# Autodesk Inventor assembly: Shooter
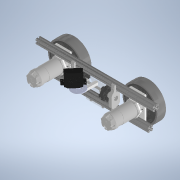
[picture p0: Inventor's stored thumbnail of the model, 180x180]
Saved by Autodesk Inventor 2021 (Build 250183000, 183)
## iProperties
Created: 2021-05-22
Part Number: Shooter
Document SubType Name: Assembly
Designer: sami8
Author: sami8
## Documents named in this file (24)
- C:\Users\sami8\Documents\FTC 2021\CAD\Shooter\Shooter.iam
- C:\Users\sami8\Documents\FTC 2021\CAD\FloorRoller\REV-41-1097.ipt
- C:\Users\sami8\Documents\FTC 2021\CAD\FloorRoller\REV-41-1363.ipt
- C:\Users\sami8\Documents\FTC 2021\CAD\Shooter\ServoArm.ipt
- C:\Users\sami8\Documents\FTC 2021\CAD\FloorRoller\REV-41-1123.ipt
- C:\Users\sami8\Documents\FTC 2021\CAD\Shooter\REV-41-1607.ipt
- C:\Users\sami8\Documents\FTC 2021\CAD\Shooter\REV-41-1608.ipt
- C:\Users\sami8\Documents\FTC 2021\CAD\Shooter\REV-41-1604.ipt
- C:\Users\sami8\Documents\FTC 2021\CAD\Shooter\REV-41-1291.ipt
- C:\Users\sami8\Documents\FTC 2021\CAD\Shooter\M3X10.ipt
- C:\Users\sami8\Documents\FTC 2021\CAD\Shooter\am-3665 4IN 5mm Hex Stealth Wheel REV2.ipt
- C:\Users\sami8\Documents\FTC 2021\CAD\Shooter\REV-41-1125.ipt
- C:\Users\sami8\Documents\FTC 2021\CAD\Shooter\FlywheelSpacer.ipt
- C:\Users\sami8\Documents\FTC 2021\CAD\Shooter\REV-41-1432.ipt
- C:\Users\sami8\Documents\FTC 2021\CAD\Shooter\MotorBracket.ipt
- C:\Users\sami8\Documents\FTC 2021\CAD\Base\REV-41-1361 Simple.ipt
- C:\Users\sami8\Documents\FTC 2021\CAD\Shooter\REV-41-1344.ipt
- C:\Users\sami8\Documents\FTC 2021\CAD\Base\REV-41-1327.ipt
- C:\Users\sami8\Documents\FTC 2021\CAD\FloorRoller\REV-41-1326.ipt
- C:\Users\sami8\Documents\FTC 2021\CAD\FloorRoller\REV-49-1559.ipt
- C:\Users\sami8\Documents\FTC 2021\CAD\Shooter\TubingHexShaft.ipt
- C:\Users\sami8\Documents\FTC 2021\CAD\Shooter\BearingBlocks.ipt
- C:\Users\sami8\Documents\FTC 2021\CAD\Shooter\PolyWedge.ipt
- C:\Users\sami8\Documents\FTC 2021\CAD\Shooter\REV-41-1432_311mm.ipt
## Components (85 placed, 23 different names)
1. REV-41-1432_311mm:2 — Flush:1, Mate:1, Flush:4, Mate:2, Mate:3, Flush:5, Mate:4, Mate:5, Mate:8, Mate:9, Flush:7
2. REV-41-1432:2 — Flush:3, Flush:6, Flush:2, Flush:7
3. REV-41-1607:3
4. REV-41-1608:3
5. REV-41-1604:3
6. REV-41-1291:3
7. M3X10:13
8. M3X10:14
9. M3X10:15
10. M3X10:16
11. M3X10:17
12. M3X10:18
13. am-3665 4IN 5mm Hex Stealth Wheel REV2:3
14. REV-41-1125:5
15. REV-41-1125:6
16. FlywheelSpacer:3
17. MotorBracket:2 — Flush:3, Flush:4, Mate:2
18. REV-41-1123:10
19. REV-41-1361 Simple:5
20. REV-41-1123:11
21. REV-41-1361 Simple:6
22. REV-41-1123:12
23. REV-41-1361 Simple:7
24. REV-41-1123:13
25. REV-41-1361 Simple:8
26. REV-41-1123:14
27. REV-41-1123:15
28. REV-41-1123:16
29. REV-41-1607:2
30. REV-41-1608:2
31. REV-41-1604:2 — Rigid:40
32. REV-41-1291:2
33. M3X10:7
34. M3X10:8
35. M3X10:9
36. M3X10:10
37. M3X10:11
38. M3X10:12
39. am-3665 4IN 5mm Hex Stealth Wheel REV2:2
40. REV-41-1125:3
41. REV-41-1125:4
42. FlywheelSpacer:2
43. MotorBracket:1 — Rigid:40, Flush:1, Mate:1, Flush:2, Rigid:42, Rigid:43, Rigid:44, Rigid:45, Rigid:46, Rigid:47, Rigid:48, Rigid:49, Rigid:50, Rigid:51, Rigid:52
44. REV-41-1123:3 — Rigid:45
45. REV-41-1361 Simple:1 — Rigid:49
46. REV-41-1123:4 — Rigid:47
47. REV-41-1361 Simple:2 — Rigid:48
48. REV-41-1123:5 — Rigid:43
49. REV-41-1361 Simple:3 — Rigid:46
50. REV-41-1123:6 — Rigid:42
51. REV-41-1361 Simple:4 — Rigid:44
52. REV-41-1123:7 — Rigid:51
53. REV-41-1123:8 — Rigid:52
54. REV-41-1123:9 — Rigid:50
55. REV-41-1097:1 — Rigid:98
56. REV-41-1363:1 — Rigid:98, Rigid:97
57. ServoArm:1 — Rigid:3, Rigid:4, Rigid:97
58. REV-41-1123:1 — Rigid:3
59. REV-41-1123:2 — Rigid:4
60. PolyWedge:1 — Mate:8, Mate:9, Rigid:101, Rigid:102, Rigid:99, Rigid:100
61. REV-41-1361 Simple:13 — Rigid:99
62. REV-41-1123:21 — Rigid:101
63. REV-41-1361 Simple:14 — Rigid:100
64. REV-41-1123:22 — Rigid:102
65. REV-41-1344:1 — Rigid:81, Rigid:83
66. REV-41-1344:2 — Rigid:82, Rigid:84
67. REV-41-1327:1 — Rigid:82
68. REV-41-1326:1 — Rigid:86
69. REV-49-1559:1 — Rigid:95
70. REV-41-1327:2 — Rigid:81
71. REV-41-1326:2 — Rigid:85
72. REV-49-1559:2 — Rigid:96
73. REV-41-1327:3 — Rigid:84
74. REV-41-1327:4 — Rigid:83
75. TubingHexShaft:1 — Rigid:85, Rigid:86
76. BearingBlocks:1 — Rigid:87, Rigid:88, Rigid:89, Rigid:90, Rigid:95, Mate:3, Flush:5, Flush:6
77. REV-41-1361 Simple:9 — Rigid:88
78. REV-41-1123:17 — Rigid:89
79. REV-41-1361 Simple:10 — Rigid:87
80. REV-41-1123:18 — Rigid:90
81. BearingBlocks:2 — Rigid:96
82. REV-41-1361 Simple:11
83. REV-41-1123:19
84. REV-41-1361 Simple:12
85. REV-41-1123:20
## Relationships (92: WeldJoint 76, Flush 7, Mate 7, RevoluteJoint 2)
- Rigid:98 [WeldJoint]: REV-41-1097:1 ↔ REV-41-1363:1
- Rigid:3 [WeldJoint]: ServoArm:1 ↔ REV-41-1123:1
- Rigid:4 [WeldJoint]: ServoArm:1 ↔ REV-41-1123:2
- [RevoluteJoint]: REV-41-1608:2 ↔ REV-41-1291:2
- [WeldJoint]: REV-41-1607:2 ↔ REV-41-1291:2
- [WeldJoint]: REV-41-1607:2 ↔ REV-41-1604:2
- [WeldJoint]: REV-41-1604:2 ↔ M3X10:12
- [WeldJoint]: REV-41-1604:2 ↔ M3X10:7
- [WeldJoint]: REV-41-1604:2 ↔ M3X10:8
- [WeldJoint]: REV-41-1604:2 ↔ M3X10:10
- [WeldJoint]: REV-41-1604:2 ↔ M3X10:9
- [WeldJoint]: REV-41-1604:2 ↔ M3X10:11
- [WeldJoint]: am-3665 4IN 5mm Hex Stealth Wheel REV2:2 ↔ REV-41-1125:3
- [WeldJoint]: am-3665 4IN 5mm Hex Stealth Wheel REV2:2 ↔ REV-41-1125:4
- [WeldJoint]: REV-41-1604:2 ↔ FlywheelSpacer:2
- [WeldJoint]: am-3665 4IN 5mm Hex Stealth Wheel REV2:2 ↔ FlywheelSpacer:2
- Rigid:40 [WeldJoint]: REV-41-1604:2 ↔ MotorBracket:1
- Flush:1: REV-41-1432_311mm:2 ↔ MotorBracket:1
- Mate:1: REV-41-1432_311mm:2 ↔ MotorBracket:1
- Flush:2 (40 mm): REV-41-1432:2 ↔ MotorBracket:1
- Rigid:42 [WeldJoint] (1.2 mm): MotorBracket:1 ↔ REV-41-1123:6
- Rigid:43 [WeldJoint] (1.2 mm): MotorBracket:1 ↔ REV-41-1123:5
- Rigid:44 [WeldJoint]: MotorBracket:1 ↔ REV-41-1361 Simple:4
- Rigid:45 [WeldJoint] (1.2 mm): MotorBracket:1 ↔ REV-41-1123:3
- Rigid:46 [WeldJoint]: MotorBracket:1 ↔ REV-41-1361 Simple:3
- Rigid:47 [WeldJoint] (1.2 mm): MotorBracket:1 ↔ REV-41-1123:4
- Rigid:48 [WeldJoint]: MotorBracket:1 ↔ REV-41-1361 Simple:2
- Rigid:49 [WeldJoint]: MotorBracket:1 ↔ REV-41-1361 Simple:1
- Rigid:50 [WeldJoint]: MotorBracket:1 ↔ REV-41-1123:9
- Rigid:51 [WeldJoint]: MotorBracket:1 ↔ REV-41-1123:7
- Rigid:52 [WeldJoint]: MotorBracket:1 ↔ REV-41-1123:8
- [RevoluteJoint]: REV-41-1608:3 ↔ REV-41-1291:3
- [WeldJoint]: REV-41-1607:3 ↔ REV-41-1291:3
- [WeldJoint]: REV-41-1607:3 ↔ REV-41-1604:3
- [WeldJoint]: REV-41-1604:3 ↔ M3X10:18
- [WeldJoint]: REV-41-1604:3 ↔ M3X10:13
- [WeldJoint]: REV-41-1604:3 ↔ M3X10:14
- [WeldJoint]: REV-41-1604:3 ↔ M3X10:16
- [WeldJoint]: REV-41-1604:3 ↔ M3X10:15
- [WeldJoint]: REV-41-1604:3 ↔ M3X10:17
- [WeldJoint]: am-3665 4IN 5mm Hex Stealth Wheel REV2:3 ↔ REV-41-1125:5
- [WeldJoint]: am-3665 4IN 5mm Hex Stealth Wheel REV2:3 ↔ REV-41-1125:6
- [WeldJoint]: REV-41-1604:3 ↔ FlywheelSpacer:3
- [WeldJoint]: am-3665 4IN 5mm Hex Stealth Wheel REV2:3 ↔ FlywheelSpacer:3
- [WeldJoint]: REV-41-1604:3 ↔ MotorBracket:2
- [WeldJoint] (1.2 mm): MotorBracket:2 ↔ REV-41-1123:13
- [WeldJoint] (1.2 mm): MotorBracket:2 ↔ REV-41-1123:12
- [WeldJoint]: MotorBracket:2 ↔ REV-41-1361 Simple:8
- [WeldJoint] (1.2 mm): MotorBracket:2 ↔ REV-41-1123:10
- [WeldJoint]: MotorBracket:2 ↔ REV-41-1361 Simple:7
- [WeldJoint] (1.2 mm): MotorBracket:2 ↔ REV-41-1123:11
- [WeldJoint]: MotorBracket:2 ↔ REV-41-1361 Simple:6
- [WeldJoint]: MotorBracket:2 ↔ REV-41-1361 Simple:5
- [WeldJoint]: MotorBracket:2 ↔ REV-41-1123:16
- [WeldJoint]: MotorBracket:2 ↔ REV-41-1123:14
- [WeldJoint]: MotorBracket:2 ↔ REV-41-1123:15
- Flush:3 (40 mm): REV-41-1432:2 ↔ MotorBracket:2
- Flush:4: REV-41-1432_311mm:2 ↔ MotorBracket:2
- Mate:2: REV-41-1432_311mm:2 ↔ MotorBracket:2
- [WeldJoint]: REV-41-1326:1 ↔ REV-49-1559:1
- [WeldJoint] (0.237 mm): REV-41-1327:1 ↔ REV-41-1326:1
- [WeldJoint]: REV-41-1326:2 ↔ REV-49-1559:2
- [WeldJoint] (0.237 mm): REV-41-1327:2 ↔ REV-41-1326:2
- Rigid:81 [WeldJoint]: REV-41-1344:1 ↔ REV-41-1327:2
- Rigid:82 [WeldJoint]: REV-41-1344:2 ↔ REV-41-1327:1
- Rigid:83 [WeldJoint]: REV-41-1344:1 ↔ REV-41-1327:4
- Rigid:84 [WeldJoint]: REV-41-1344:2 ↔ REV-41-1327:3
- Rigid:85 [WeldJoint]: REV-41-1326:2 ↔ TubingHexShaft:1
- Rigid:86 [WeldJoint]: REV-41-1326:1 ↔ TubingHexShaft:1
- Rigid:87 [WeldJoint]: BearingBlocks:1 ↔ REV-41-1361 Simple:10
- Rigid:88 [WeldJoint]: BearingBlocks:1 ↔ REV-41-1361 Simple:9
- Rigid:89 [WeldJoint] (-1.2 mm): BearingBlocks:1 ↔ REV-41-1123:17
- Rigid:90 [WeldJoint] (-1.2 mm): BearingBlocks:1 ↔ REV-41-1123:18
- [WeldJoint]: BearingBlocks:2 ↔ REV-41-1361 Simple:12
- [WeldJoint]: BearingBlocks:2 ↔ REV-41-1361 Simple:11
- [WeldJoint] (-1.2 mm): BearingBlocks:2 ↔ REV-41-1123:19
- [WeldJoint] (-1.2 mm): BearingBlocks:2 ↔ REV-41-1123:20
- Rigid:95 [WeldJoint]: REV-49-1559:1 ↔ BearingBlocks:1
- Rigid:96 [WeldJoint]: REV-49-1559:2 ↔ BearingBlocks:2
- Mate:3: REV-41-1432_311mm:2 ↔ BearingBlocks:1
- Flush:5: REV-41-1432_311mm:2 ↔ BearingBlocks:1
- Flush:6 (108 mm): REV-41-1432:2 ↔ BearingBlocks:1
- Mate:4: REV-41-1432_311mm:2
- Mate:5: REV-41-1432_311mm:2
- Rigid:97 [WeldJoint]: REV-41-1363:1 ↔ ServoArm:1
- Mate:8: REV-41-1432_311mm:2 ↔ PolyWedge:1
- Mate:9 (3 mm): REV-41-1432_311mm:2 ↔ PolyWedge:1
- Rigid:101 [WeldJoint] (-1.2 mm): PolyWedge:1 ↔ REV-41-1123:21
- Rigid:102 [WeldJoint] (-1.2 mm): PolyWedge:1 ↔ REV-41-1123:22
- Rigid:99 [WeldJoint]: PolyWedge:1 ↔ REV-41-1361 Simple:13
- Rigid:100 [WeldJoint]: PolyWedge:1 ↔ REV-41-1361 Simple:14
- Flush:7 (15 mm): REV-41-1432_311mm:2 ↔ REV-41-1432:2
## Named parameters: d29_d18 = 0 mm, d30_d19 = 0 mm, d39_d4 = 0 mm, d40_d5 = -150.867512 deg, d41_d6 = 0 mm, d42_d7 = 0 mm, d43_d8 = 0 mm, d44_d9 = 0 mm, d45_d10 = 0 mm, d46_d11 = 0 mm, d47_d12 = 0 mm, d48_d13 = 0 mm, d49_d15 = 0 mm, d50_d16 = 0 mm, d69_d29_d18 = 0 mm, d70_d30_d19 = 0 mm, d71_d39_d4 = 0 mm, d72_d40_d5 = -150.873724 deg, d73_d41_d6 = 0 mm, d74_d42_d7 = 0 mm, d75_d43_d8 = 0 mm, d76_d44_d9 = 0 mm, d77_d45_d10 = 0 mm, d78_d46_d11 = 0 mm, d79_d47_d12 = 0 mm, d80_d48_d13 = 0 mm, d81_d49_d15 = 0 mm, d82_d50_d16 = 0 mm, d83_d51 = 0 mm, d84_d58 = 1.2 mm, d85_d59 = 1.2 mm, d86_d60 = 0 mm, d87_d61 = 1.2 mm, d88_d62 = 0 mm, d89_d63 = 1.2 mm, d90_d64 = 0 mm, d91_d65 = 0 mm, d92_d66 = 0 mm, d93_d67 = 0 mm, d94_d68 = 0 mm, d57_d20 = 0 mm, d103_d60 = 0.237 mm, d104_d57_d20 = 0 mm, d105_d103_d60 = 0.237 mm, d116_d112 = 0 mm, d117_d113 = 0 mm, d118_d114 = -1.2 mm, d119_d115 = -1.2 mm
